# Autodesk Inventor assembly: Unwrap
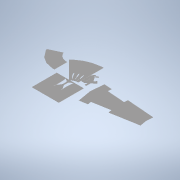
[picture p0: Inventor's stored thumbnail of the model, 180x180]
Saved by Autodesk Inventor 2020 (Build 240168000, 168)
## iProperties
Created: 2020-03-11
Part Number: Unwrap
Document SubType Name: Assembly
Designer: valem
Author: valem
## Documents named in this file (8)
- D:\Planes\Cardboard_glider_1\Unwrap.iam
- D:\Planes\Cardboard_glider_1\Unwrap_wing_1.ipt
- D:\Planes\Cardboard_glider_1\nose_cap_1.ipt
- D:\Planes\Cardboard_glider_1\Cabin_1.ipt
- D:\Planes\Cardboard_glider_1\Main body_1.ipt
- D:\Planes\Cardboard_glider_1\Tail_1.ipt
- D:\Planes\Cardboard_glider_1\Solid3.ipt
- D:\Planes\Cardboard_glider_1\Solid3_1.ipt
## Components (7 placed, 7 different names)
1. Unwrap_wing_1:1 — Mate:2
2. nose_cap_1:1 — Mate:4
3. Cabin_1:1 — Mate:5
4. Main body_1:1 — Mate:6
5. Tail_1:1 — Mate:7
6. Solid3:1 — Mate:3
7. Solid3_1:1 — Mate:1
## Relationships (7: Mate 7)
- Mate:1: Solid3_1:1
- Mate:2: Unwrap_wing_1:1
- Mate:3: Solid3:1
- Mate:4: nose_cap_1:1
- Mate:5: Cabin_1:1
- Mate:6: Main body_1:1
- Mate:7: Tail_1:1
